# Autodesk Inventor assembly: CJ2KB10-75Z(0_1_0)
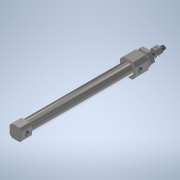
[picture p0: Inventor's stored thumbnail of the model, 180x180]
Saved by Autodesk Inventor 2022.3 (Build 263350000, 350)
## iProperties
Category: PARTsolutions
Company: SMC
Created: 2019-10-24
Part Number: CJ2KB10-75Z(0_1_0)
Catalog Web Link: www.cadenas.de
Description: CJ2K-Z/CDJ2K-Z-Air Cylinder/Non-rotating Rod Type: Double Acting, Single Rod
Vendor: SMC
Document SubType Name: Assembly
Designer: psadmin
Manufacturer: SMC
Mass: 78.7892 g
Surface Area: 110.206 cm^2
Volume: 9.84865 cm^3
PSOL_IDENT_0: {$CADENAS_DATA\23d-libs\smc_jp\actuator\standard_air_cylinder\cj2\cj2k_z_asmtab.prj},303 {VTYP=3D},{
PSOL_IDENT_1: STYP=ASSTAB},{NB=CJ2KB10-75Z(0_1_0)},{LINA=CJ2KB10-75Z},{NN=CJ2K-Z/CDJ2K-Z},{DATE=07.02.2019 07:32:0
PSOL_IDENT_2: 1},{GEOMDATE=08.08.2017 00:58:17},{VERSION=},{LINEID=370},{WBVAR=MAGNET,AUTOSWITCH,LEAD,NUMBER,STROK
PSOL_IDENT_3: E,POS,PORT,STOP,BRACKET,RODB,MOUNTING,OMSC,OMSCXC3,OMSCXC51,THREAD},{WBNUMERIC=STROKE,POS}  {NB=CJ2K
PSOL_IDENT_4: B10-75Z(0_1_0)},{LINA=CJ2KB10-75Z},{KT=DUMMY},{ORDER=CJ2KB10-75Z},{BORE=10},{MOUNT=(B) Basic},{MOUNT
PSOL_IDENT_5: X=B},{MAGNET=},{AUTOSWITCH=},{AUTOSWX='','N/A'},{LEAD=},{LEADX= '','N/A' },{NUMBER=},{SWSIGNX= '','N
PSOL_IDENT_6: /A' },{STROKE=75},{STDSTROKE=15,30,45,60,75,100,125,150},{STROKE1X=[2:150/1]},{SMIN=2},{SMINASW1=10}
PSOL_IDENT_7: ,{SMINASW2=15},{SMAX=150},{POS=0},{PORT=},{PORTX='', '(-) Perpendicular', 'R', '(R) In-line'},{STOP=
PSOL_IDENT_8: 1},{COM=Please confirm the conditions of use with SMC},{BRACKET=},{RODB=},{MOUNTING=},{MOUNTINGX='','
PSOL_IDENT_9: N/A'},{OMSC=},{OMSCXC3=},{OMSCXC51=},{THREAD=0},{SW=B},{PPATH=cj2k_z/assembly/cj2k_z_asmsbl.prj},{MO
PSOL_IDENT_10: DEL=CJ2KB10-75Z},{NENN=CJ2KB10-75Z},{BRACKETX='','N/A'},{XC3= '','(-) None','-XC3AB','(XC3AB) Specia
PSOL_IDENT_11: l Port Location (Rod port location: A,Head port location: B)','-XC3AC','(XC3AC) Special Port Locatio
PSOL_IDENT_12: n (Rod port location: A,Head port location: C)','-XC3AD','(XC3AD) Special Port Location (Rod port lo
PSOL_IDENT_13: cation : A,Head port location: D)','-XC3BA','(XC3BA) Special Port Location (Rod port location: B,Hea
PSOL_IDENT_14: d port location: A)','-XC3BB','(XC3BB) Special Port Location (Rod port location: B,Head port locatio
PSOL_IDENT_15: n viewed: B)','-XC3BC','(XC3BC) Special Port Location (Rod port location: B,Head port location: C)','
PSOL_IDENT_16: -XC3BD','(XC3BD) Special Port Location (Rod port location: B,Head port location: D)','-XC3CA','(XC3C
PSOL_IDENT_17: A) Special Port Location (Rod port location: C,Head port location: A)','-XC3CB','(XC3CB) Special Por
PSOL_IDENT_18: t Location (Rod port location: C,Head port location: B)','-XC3CC','(XC3CC) Special Port Location (Ro
PSOL_IDENT_19: d port location: C,Head port location: C)','-XC3CD','(XC3CD) Special Port Location (Rod port locatio
PSOL_IDENT_20: n: C,Head port location: D)','-XC3DA','(XC3DA) Special Port Location (Rod port location: D,Head port
PSOL_IDENT_21: location: A)','-XC3DB','(XC3DB) Special Port Location (Rod port location: D,Head port location: B)'
PSOL_IDENT_22: ,'-XC3DC','(XC3DC) Special Port Location (Rod port location: D,Head port location: C)','-XC3DD','(XC
PSOL_IDENT_23: 3DD) Special Port Location (Rod port location: D,Head port location: D)' },{XC51= '','(-) None','-XC
PSOL_IDENT_24: 51H4','(XC51H4) Hose nipple type: ø4/2.5 with restriction','-XC51H6','(XC51H6) Hose nipple type: ø6/
PSOL_IDENT_25: 4 with restriction','-XC51MH4','(XC51MH4) Hose nipple type: ø4/2.5 without restriction','-XC51MH6','
PSOL_IDENT_26: (XC51MH6) Hose nipple type: ø6/4 without restriction' },{OMSCX= '', '(-) None', '-XC22', '(XC22) Flu
PSOL_IDENT_27: ororubber seals', '-XC85'  , '(XC85) Grease specification for food processing machines', '-X446'  , '
PSOL_IDENT_28: (X446) PTFE grease' }
NN: CJ2K-Z/CDJ2K-Z
NT: Air Cylinder/Non-rotating Rod Type: Double Acting, Single Rod
NB: CJ2KB10-75Z(0_1_0)
NBSYN: $ORDER.($POS._$STOP._$THREAD.)
LINA: CJ2KB10-75Z
ROWDESC: CJ2KB10-75Z
BORE: 10
MOUNT: (B) Basic
MAGNET: (-) Without magnet
AUTOSWITCH: N/A
LEAD: N/A
NUMBER: N/A
STROKE: 75
POS: 0
PORT: (-) Perpendicular
STOP: Manufacturable stroke
COM: Please confirm the conditions of use with SMC
BRACKET: N/A
RODB: (-) None
MOUNTING: N/A
OMSC: (-) None
OMSCXC3: (-) None
OMSCXC51: (-) None
THREAD: on
SUPPLIER: SMC
ARTICLENO: CJ2KB10-75Z(0_1_0)
BOMINFO: CJ2KB10-75Z
CREATOR: CADENAS GmbH
Title: CJ2KB10-75Z
Author: Cadenas PARTsolutions
Comments: Air Cylinder/Non-rotating Rod Type: Double Acting, Single Rod
## Documents named in this file (5)
- C:\Users\YusukeKunita\Documents\GrabCAD\Development\BasicParts\AirCylinder\CJ2KB10-75Z\CJ2KB10-75Z.iam
- C:\Users\YusukeKunita\Documents\GrabCAD\Development\BasicParts\AirCylinder\CJ2KB10-75Z\CJ2KB10-75Z_BODY.ipt
- C:\Users\YusukeKunita\Documents\GrabCAD\Development\BasicParts\AirCylinder\CJ2KB10-75Z\CJ2K10Z_NUT.ipt
- C:\Users\YusukeKunita\Documents\GrabCAD\Development\BasicParts\AirCylinder\CJ2KB10-75Z\CJ2KB10-75Z_ROD.ipt
- C:\Users\YusukeKunita\Documents\GrabCAD\Development\BasicParts\AirCylinder\CJ2KB10-75Z\NTJ-010C.ipt
## Components (5 placed, 4 different names)
1. CJ2KB10-75Z_BODY:1 — body_XY@1 <-> NUT_XY@2, body_Z@1 <-> NUT_Z@2, body_YZ@1 <-> NUT_YZ@2, rod_Z@1 <-> rod_Z@3, rod_YZ@1 <-> rod_YZ@3, メイト:8
2. CJ2K10Z_NUT:1 — body_XY@1 <-> NUT_XY@2, body_Z@1 <-> NUT_Z@2, body_YZ@1 <-> NUT_YZ@2
3. CJ2KB10-75Z_ROD:1 — rod_Z@1 <-> rod_Z@3, rod_YZ@1 <-> rod_YZ@3, rodnt1_XY@3 <-> ntj_XY@4, rodnt1_Z@3 <-> ntj_Z@4, rodnt1_YZ@3 <-> ntj_YZ@4, rodnt2_XY@3 <-> ntj_XY@5, rodnt2_Z@3 <-> ntj_Z@5, rodnt2_YZ@3 <-> ntj_YZ@5
4. NTJ-010C:1 — rodnt1_XY@3 <-> ntj_XY@4, rodnt1_Z@3 <-> ntj_Z@4, rodnt1_YZ@3 <-> ntj_YZ@4, メイト:8
5. NTJ-010C:2 — rodnt2_XY@3 <-> ntj_XY@5, rodnt2_Z@3 <-> ntj_Z@5, rodnt2_YZ@3 <-> ntj_YZ@5
## Relationships (12: Mate 8, Angle 4)
- body_XY@1 <-> NUT_XY@2 [Mate] (-2.3 mm): CJ2KB10-75Z_BODY:1 ↔ CJ2K10Z_NUT:1
- body_Z@1 <-> NUT_Z@2 [Mate]: CJ2KB10-75Z_BODY:1 ↔ CJ2K10Z_NUT:1
- body_YZ@1 <-> NUT_YZ@2 [Angle] (0 deg): CJ2KB10-75Z_BODY:1 ↔ CJ2K10Z_NUT:1
- rod_Z@1 <-> rod_Z@3 [Mate]: CJ2KB10-75Z_BODY:1 ↔ CJ2KB10-75Z_ROD:1
- rod_YZ@1 <-> rod_YZ@3 [Angle] (0 deg): CJ2KB10-75Z_BODY:1 ↔ CJ2KB10-75Z_ROD:1
- rodnt1_XY@3 <-> ntj_XY@4 [Mate]: CJ2KB10-75Z_ROD:1 ↔ NTJ-010C:1
- rodnt1_Z@3 <-> ntj_Z@4 [Mate]: CJ2KB10-75Z_ROD:1 ↔ NTJ-010C:1
- rodnt1_YZ@3 <-> ntj_YZ@4 [Angle] (0 deg): CJ2KB10-75Z_ROD:1 ↔ NTJ-010C:1
- rodnt2_XY@3 <-> ntj_XY@5 [Mate]: CJ2KB10-75Z_ROD:1 ↔ NTJ-010C:2
- rodnt2_Z@3 <-> ntj_Z@5 [Mate]: CJ2KB10-75Z_ROD:1 ↔ NTJ-010C:2
- rodnt2_YZ@3 <-> ntj_YZ@5 [Angle] (0 deg): CJ2KB10-75Z_ROD:1 ↔ NTJ-010C:2
- メイト:8 [Mate] (4 mm): CJ2KB10-75Z_BODY:1 ↔ NTJ-010C:1
